# Autodesk Inventor assembly: Stadio6
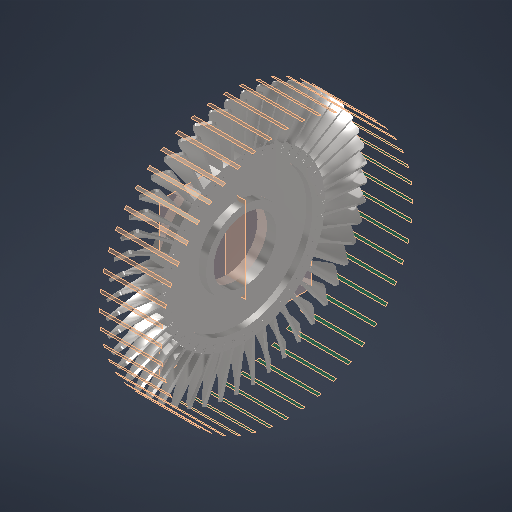
[picture p0: Inventor's stored thumbnail of the model, 512x512]
Saved by Autodesk Inventor 2026.2 (Build 302298010, 298A)
## iProperties
Created: 2026-04-24
Part Number: Stadio6
Document SubType Name: Assembly
Designer: Yan
Author: Yan
## Documents named in this file (3)
- C:\Users\Yan\Desktop\Turbina\Stadio6.iam
- C:\Users\Yan\Desktop\Turbina\DiscoPaleStadio6-DimensioniAprossimate.ipt
- C:\Users\Yan\Desktop\Turbina\PalaStadio6.ipt
## Components (49 placed, 2 different names)
1. DiscoPaleStadio6-DimensioniAprossimate:1 — Mate:1, Mate:2, Mate:3, Mate:4, Mate:5, Mate:6, Mate:7, Mate:8, Mate:9, Mate:10, Mate:11, Mate:12, Mate:13, Mate:14, Mate:15, Mate:16, Mate:17, Mate:18, Mate:19, Mate:20, Mate:21, Mate:22, Mate:24, Mate:25, Mate:26, Mate:27, Mate:28, Mate:29, Mate:30, Mate:31, Mate:32, Mate:33, Mate:34, Mate:35, Mate:36, Mate:37, Mate:38, Mate:39, Mate:40, Mate:41, Mate:42, Mate:43, Mate:44, Mate:45, Mate:46, Mate:47, Mate:48, Mate:49, Mate:50, Mate:51, Mate:52, Mate:53, Mate:56, Mate:57, Mate:58, Mate:59, Mate:60, Mate:61, Mate:62, Mate:63, Mate:64, Mate:65, Mate:66, Mate:67, Mate:68, Mate:69, Mate:70, Mate:71, Mate:72, Mate:73, Mate:74, Mate:75, Mate:76, Mate:77, Mate:78, Mate:79, Mate:80, Mate:81, Mate:82, Mate:83, Mate:84, Mate:85, Mate:86, Mate:87, Mate:88, Mate:89, Mate:90, Mate:91, Mate:92, Mate:93, Mate:94, Mate:95, Mate:96, Mate:97, Mate:98, Flush:1, Flush:2, Flush:3, Flush:4, Flush:5, Flush:6, Flush:7, Flush:8, Flush:9, Flush:10, Flush:11, Flush:12, Flush:13, Flush:14, Flush:15, Flush:16, Flush:17, Flush:18, Flush:19, Flush:20, Flush:21, Flush:22, Flush:23, Flush:24, Flush:25, Flush:26, Flush:27, Flush:28, Flush:29, Flush:30, Flush:31, Flush:32, Flush:33, Flush:34, Flush:35, Flush:36, Flush:37, Flush:38, Flush:39, Flush:40, Flush:41, Flush:42, Flush:43, Flush:44, Flush:45, Flush:46, Flush:47, Flush:48, Mate:99, Mate:100
2. PalaStadio6:1 — Mate:1, Mate:28, Flush:30
3. PalaStadio6:2 — Mate:2, Mate:27, Flush:29
4. PalaStadio6:3 — Mate:3, Mate:76, Mate:77, Flush:28
5. PalaStadio6:4 — Mate:4, Mate:29, Flush:27
6. PalaStadio6:5 — Mate:5, Mate:30, Flush:26
7. PalaStadio6:6 — Mate:7, Mate:32, Flush:24
8. PalaStadio6:7 — Mate:8, Mate:33, Flush:23
9. PalaStadio6:8 — Mate:9, Mate:34, Flush:22
10. PalaStadio6:9 — Mate:10, Mate:35, Flush:21
11. PalaStadio6:10 — Mate:11, Mate:36, Flush:20
12. PalaStadio6:11 — Mate:12, Mate:37, Flush:19
13. PalaStadio6:12 — Mate:13, Mate:38, Flush:18
14. PalaStadio6:13 — Mate:68, Mate:81, Flush:36
15. PalaStadio6:14 — Mate:6, Mate:31, Flush:25
16. PalaStadio6:15 — Mate:48, Mate:49, Flush:8
17. PalaStadio6:16 — Mate:22, Mate:47, Flush:9
18. PalaStadio6:17 — Mate:21, Mate:46, Flush:10
19. PalaStadio6:18 — Mate:20, Mate:45, Flush:11
20. PalaStadio6:19 — Mate:19, Mate:44, Flush:12
21. PalaStadio6:20 — Mate:18, Mate:43, Flush:13
22. PalaStadio6:21 — Mate:17, Mate:42, Flush:14
23. PalaStadio6:22 — Mate:16, Mate:41, Flush:15
24. PalaStadio6:23 — Mate:15, Mate:40, Flush:16
25. PalaStadio6:24 — Mate:14, Mate:39, Flush:17
26. PalaStadio6:25 — Mate:60, Mate:91, Flush:45
27. PalaStadio6:26 — Mate:59, Mate:92, Flush:46
28. PalaStadio6:27 — Mate:87, Flush:42
29. PalaStadio6:28 — Mate:58, Mate:93, Flush:47
30. PalaStadio6:29 — Mate:57, Mate:94, Flush:48
31. PalaStadio6:30 — Mate:56, Mate:95, Flush:2
32. PalaStadio6:31 — Mate:97, Flush:1, Mate:100
33. PalaStadio6:32 — Mate:98, Flush:3, Mate:99
34. PalaStadio6:33 — Mate:53, Mate:96, Flush:4
35. PalaStadio6:34 — Mate:26, Mate:52, Flush:5
36. PalaStadio6:35 — Mate:25, Mate:51, Flush:6
37. PalaStadio6:36 — Mate:24, Mate:50, Flush:7
38. PalaStadio6:37 — Mate:72, Mate:75, Flush:32
39. PalaStadio6:38 — Mate:73, Mate:74, Flush:31
40. PalaStadio6:39 — Mate:70, Mate:79, Flush:34
41. PalaStadio6:40 — Mate:71, Mate:78, Flush:33
42. PalaStadio6:41 — Mate:69, Mate:80, Flush:35
43. PalaStadio6:42 — Mate:67, Mate:82, Flush:37
44. PalaStadio6:43 — Mate:66, Mate:83, Flush:38
45. PalaStadio6:44 — Mate:65, Mate:84, Flush:39
46. PalaStadio6:45 — Mate:64, Mate:85, Mate:88, Flush:40
47. PalaStadio6:46 — Mate:63, Mate:86, Flush:41
48. PalaStadio6:47 — Mate:62, Mate:89, Flush:43
49. PalaStadio6:48 — Mate:61, Mate:90, Flush:44
## Relationships (145: Mate 97, Flush 48)
- Mate:1: DiscoPaleStadio6-DimensioniAprossimate:1 ↔ PalaStadio6:1
- Mate:2: DiscoPaleStadio6-DimensioniAprossimate:1 ↔ PalaStadio6:2
- Mate:3: DiscoPaleStadio6-DimensioniAprossimate:1 ↔ PalaStadio6:3
- Mate:4: DiscoPaleStadio6-DimensioniAprossimate:1 ↔ PalaStadio6:4
- Mate:5: DiscoPaleStadio6-DimensioniAprossimate:1 ↔ PalaStadio6:5
- Mate:6: DiscoPaleStadio6-DimensioniAprossimate:1 ↔ PalaStadio6:14
- Mate:7: DiscoPaleStadio6-DimensioniAprossimate:1 ↔ PalaStadio6:6
- Mate:8: DiscoPaleStadio6-DimensioniAprossimate:1 ↔ PalaStadio6:7
- Mate:9: DiscoPaleStadio6-DimensioniAprossimate:1 ↔ PalaStadio6:8
- Mate:10: DiscoPaleStadio6-DimensioniAprossimate:1 ↔ PalaStadio6:9
- Mate:11: DiscoPaleStadio6-DimensioniAprossimate:1 ↔ PalaStadio6:10
- Mate:12: DiscoPaleStadio6-DimensioniAprossimate:1 ↔ PalaStadio6:11
- Mate:13: DiscoPaleStadio6-DimensioniAprossimate:1 ↔ PalaStadio6:12
- Mate:14: DiscoPaleStadio6-DimensioniAprossimate:1 ↔ PalaStadio6:24
- Mate:15: DiscoPaleStadio6-DimensioniAprossimate:1 ↔ PalaStadio6:23
- Mate:16: DiscoPaleStadio6-DimensioniAprossimate:1 ↔ PalaStadio6:22
- Mate:17: DiscoPaleStadio6-DimensioniAprossimate:1 ↔ PalaStadio6:21
- Mate:18: DiscoPaleStadio6-DimensioniAprossimate:1 ↔ PalaStadio6:20
- Mate:19: DiscoPaleStadio6-DimensioniAprossimate:1 ↔ PalaStadio6:19
- Mate:20: DiscoPaleStadio6-DimensioniAprossimate:1 ↔ PalaStadio6:18
- Mate:21: DiscoPaleStadio6-DimensioniAprossimate:1 ↔ PalaStadio6:17
- Mate:22: DiscoPaleStadio6-DimensioniAprossimate:1 ↔ PalaStadio6:16
- Mate:24: DiscoPaleStadio6-DimensioniAprossimate:1 ↔ PalaStadio6:36
- Mate:25: DiscoPaleStadio6-DimensioniAprossimate:1 ↔ PalaStadio6:35
- Mate:26: DiscoPaleStadio6-DimensioniAprossimate:1 ↔ PalaStadio6:34
- Mate:27: DiscoPaleStadio6-DimensioniAprossimate:1 ↔ PalaStadio6:2
- Mate:28: DiscoPaleStadio6-DimensioniAprossimate:1 ↔ PalaStadio6:1
- Mate:29: DiscoPaleStadio6-DimensioniAprossimate:1 ↔ PalaStadio6:4
- Mate:30: DiscoPaleStadio6-DimensioniAprossimate:1 ↔ PalaStadio6:5
- Mate:31: DiscoPaleStadio6-DimensioniAprossimate:1 ↔ PalaStadio6:14
- Mate:32: DiscoPaleStadio6-DimensioniAprossimate:1 ↔ PalaStadio6:6
- Mate:33: DiscoPaleStadio6-DimensioniAprossimate:1 ↔ PalaStadio6:7
- Mate:34: DiscoPaleStadio6-DimensioniAprossimate:1 ↔ PalaStadio6:8
- Mate:35: DiscoPaleStadio6-DimensioniAprossimate:1 ↔ PalaStadio6:9
- Mate:36: DiscoPaleStadio6-DimensioniAprossimate:1 ↔ PalaStadio6:10
- Mate:37: DiscoPaleStadio6-DimensioniAprossimate:1 ↔ PalaStadio6:11
- Mate:38: DiscoPaleStadio6-DimensioniAprossimate:1 ↔ PalaStadio6:12
- Mate:39: DiscoPaleStadio6-DimensioniAprossimate:1 ↔ PalaStadio6:24
- Mate:40: DiscoPaleStadio6-DimensioniAprossimate:1 ↔ PalaStadio6:23
- Mate:41: DiscoPaleStadio6-DimensioniAprossimate:1 ↔ PalaStadio6:22
- Mate:42: DiscoPaleStadio6-DimensioniAprossimate:1 ↔ PalaStadio6:21
- Mate:43: DiscoPaleStadio6-DimensioniAprossimate:1 ↔ PalaStadio6:20
- Mate:44: DiscoPaleStadio6-DimensioniAprossimate:1 ↔ PalaStadio6:19
- Mate:45: DiscoPaleStadio6-DimensioniAprossimate:1 ↔ PalaStadio6:18
- Mate:46: DiscoPaleStadio6-DimensioniAprossimate:1 ↔ PalaStadio6:17
- Mate:47: DiscoPaleStadio6-DimensioniAprossimate:1 ↔ PalaStadio6:16
- Mate:48: DiscoPaleStadio6-DimensioniAprossimate:1 ↔ PalaStadio6:15
- Mate:49: DiscoPaleStadio6-DimensioniAprossimate:1 ↔ PalaStadio6:15
- Mate:50: DiscoPaleStadio6-DimensioniAprossimate:1 ↔ PalaStadio6:36
- Mate:51: DiscoPaleStadio6-DimensioniAprossimate:1 ↔ PalaStadio6:35
- Mate:52: DiscoPaleStadio6-DimensioniAprossimate:1 ↔ PalaStadio6:34
- Mate:53: DiscoPaleStadio6-DimensioniAprossimate:1 ↔ PalaStadio6:33
- Mate:56: DiscoPaleStadio6-DimensioniAprossimate:1 ↔ PalaStadio6:30
- Mate:57: DiscoPaleStadio6-DimensioniAprossimate:1 ↔ PalaStadio6:29
- Mate:58: DiscoPaleStadio6-DimensioniAprossimate:1 ↔ PalaStadio6:28
- Mate:59: DiscoPaleStadio6-DimensioniAprossimate:1 ↔ PalaStadio6:26
- Mate:60: DiscoPaleStadio6-DimensioniAprossimate:1 ↔ PalaStadio6:25
- Mate:61: DiscoPaleStadio6-DimensioniAprossimate:1 ↔ PalaStadio6:48
- Mate:62: DiscoPaleStadio6-DimensioniAprossimate:1 ↔ PalaStadio6:47
- Mate:63: DiscoPaleStadio6-DimensioniAprossimate:1 ↔ PalaStadio6:46
- Mate:64: DiscoPaleStadio6-DimensioniAprossimate:1 ↔ PalaStadio6:45
- Mate:65: DiscoPaleStadio6-DimensioniAprossimate:1 ↔ PalaStadio6:44
- Mate:66: DiscoPaleStadio6-DimensioniAprossimate:1 ↔ PalaStadio6:43
- Mate:67: DiscoPaleStadio6-DimensioniAprossimate:1 ↔ PalaStadio6:42
- Mate:68: DiscoPaleStadio6-DimensioniAprossimate:1 ↔ PalaStadio6:13
- Mate:69: DiscoPaleStadio6-DimensioniAprossimate:1 ↔ PalaStadio6:41
- Mate:70: DiscoPaleStadio6-DimensioniAprossimate:1 ↔ PalaStadio6:39
- Mate:71: DiscoPaleStadio6-DimensioniAprossimate:1 ↔ PalaStadio6:40
- Mate:72: DiscoPaleStadio6-DimensioniAprossimate:1 ↔ PalaStadio6:37
- Mate:73: DiscoPaleStadio6-DimensioniAprossimate:1 ↔ PalaStadio6:38
- Mate:74: DiscoPaleStadio6-DimensioniAprossimate:1 ↔ PalaStadio6:38
- Mate:75: DiscoPaleStadio6-DimensioniAprossimate:1 ↔ PalaStadio6:37
- Mate:76: DiscoPaleStadio6-DimensioniAprossimate:1 ↔ PalaStadio6:3
- Mate:77: DiscoPaleStadio6-DimensioniAprossimate:1 ↔ PalaStadio6:3
- Mate:78: DiscoPaleStadio6-DimensioniAprossimate:1 ↔ PalaStadio6:40
- Mate:79: DiscoPaleStadio6-DimensioniAprossimate:1 ↔ PalaStadio6:39
- Mate:80: DiscoPaleStadio6-DimensioniAprossimate:1 ↔ PalaStadio6:41
- Mate:81: DiscoPaleStadio6-DimensioniAprossimate:1 ↔ PalaStadio6:13
- Mate:82: DiscoPaleStadio6-DimensioniAprossimate:1 ↔ PalaStadio6:42
- Mate:83: DiscoPaleStadio6-DimensioniAprossimate:1 ↔ PalaStadio6:43
- Mate:84: DiscoPaleStadio6-DimensioniAprossimate:1 ↔ PalaStadio6:44
- Mate:85: DiscoPaleStadio6-DimensioniAprossimate:1 ↔ PalaStadio6:45
- Mate:86: DiscoPaleStadio6-DimensioniAprossimate:1 ↔ PalaStadio6:46
- Mate:87: DiscoPaleStadio6-DimensioniAprossimate:1 ↔ PalaStadio6:27
- Mate:88: DiscoPaleStadio6-DimensioniAprossimate:1 ↔ PalaStadio6:45
- Mate:89: DiscoPaleStadio6-DimensioniAprossimate:1 ↔ PalaStadio6:47
- Mate:90: DiscoPaleStadio6-DimensioniAprossimate:1 ↔ PalaStadio6:48
- Mate:91: DiscoPaleStadio6-DimensioniAprossimate:1 ↔ PalaStadio6:25
- Mate:92: DiscoPaleStadio6-DimensioniAprossimate:1 ↔ PalaStadio6:26
- Mate:93: DiscoPaleStadio6-DimensioniAprossimate:1 ↔ PalaStadio6:28
- Mate:94: DiscoPaleStadio6-DimensioniAprossimate:1 ↔ PalaStadio6:29
- Mate:95: DiscoPaleStadio6-DimensioniAprossimate:1 ↔ PalaStadio6:30
- Mate:96: DiscoPaleStadio6-DimensioniAprossimate:1 ↔ PalaStadio6:33
- Mate:97: DiscoPaleStadio6-DimensioniAprossimate:1 ↔ PalaStadio6:31
- Mate:98: DiscoPaleStadio6-DimensioniAprossimate:1 ↔ PalaStadio6:32
- Flush:1: DiscoPaleStadio6-DimensioniAprossimate:1 ↔ PalaStadio6:31
- Flush:2: DiscoPaleStadio6-DimensioniAprossimate:1 ↔ PalaStadio6:30
- Flush:3: DiscoPaleStadio6-DimensioniAprossimate:1 ↔ PalaStadio6:32
- Flush:4: DiscoPaleStadio6-DimensioniAprossimate:1 ↔ PalaStadio6:33
- Flush:5: DiscoPaleStadio6-DimensioniAprossimate:1 ↔ PalaStadio6:34
- Flush:6: DiscoPaleStadio6-DimensioniAprossimate:1 ↔ PalaStadio6:35
- Flush:7: DiscoPaleStadio6-DimensioniAprossimate:1 ↔ PalaStadio6:36
- Flush:8: DiscoPaleStadio6-DimensioniAprossimate:1 ↔ PalaStadio6:15
- Flush:9: DiscoPaleStadio6-DimensioniAprossimate:1 ↔ PalaStadio6:16
- Flush:10: DiscoPaleStadio6-DimensioniAprossimate:1 ↔ PalaStadio6:17
- Flush:11: DiscoPaleStadio6-DimensioniAprossimate:1 ↔ PalaStadio6:18
- Flush:12: DiscoPaleStadio6-DimensioniAprossimate:1 ↔ PalaStadio6:19
- Flush:13: DiscoPaleStadio6-DimensioniAprossimate:1 ↔ PalaStadio6:20
- Flush:14: DiscoPaleStadio6-DimensioniAprossimate:1 ↔ PalaStadio6:21
- Flush:15: DiscoPaleStadio6-DimensioniAprossimate:1 ↔ PalaStadio6:22
- Flush:16: DiscoPaleStadio6-DimensioniAprossimate:1 ↔ PalaStadio6:23
- Flush:17: DiscoPaleStadio6-DimensioniAprossimate:1 ↔ PalaStadio6:24
- Flush:18: DiscoPaleStadio6-DimensioniAprossimate:1 ↔ PalaStadio6:12
- Flush:19: DiscoPaleStadio6-DimensioniAprossimate:1 ↔ PalaStadio6:11
- Flush:20: DiscoPaleStadio6-DimensioniAprossimate:1 ↔ PalaStadio6:10
- Flush:21: DiscoPaleStadio6-DimensioniAprossimate:1 ↔ PalaStadio6:9
- Flush:22: DiscoPaleStadio6-DimensioniAprossimate:1 ↔ PalaStadio6:8
- Flush:23: DiscoPaleStadio6-DimensioniAprossimate:1 ↔ PalaStadio6:7
- Flush:24: DiscoPaleStadio6-DimensioniAprossimate:1 ↔ PalaStadio6:6
- Flush:25: DiscoPaleStadio6-DimensioniAprossimate:1 ↔ PalaStadio6:14
- Flush:26: DiscoPaleStadio6-DimensioniAprossimate:1 ↔ PalaStadio6:5
- Flush:27: DiscoPaleStadio6-DimensioniAprossimate:1 ↔ PalaStadio6:4
- Flush:28: DiscoPaleStadio6-DimensioniAprossimate:1 ↔ PalaStadio6:3
- Flush:29: DiscoPaleStadio6-DimensioniAprossimate:1 ↔ PalaStadio6:2
- Flush:30: DiscoPaleStadio6-DimensioniAprossimate:1 ↔ PalaStadio6:1
- Flush:31: DiscoPaleStadio6-DimensioniAprossimate:1 ↔ PalaStadio6:38
- Flush:32: DiscoPaleStadio6-DimensioniAprossimate:1 ↔ PalaStadio6:37
- Flush:33: DiscoPaleStadio6-DimensioniAprossimate:1 ↔ PalaStadio6:40
- Flush:34: DiscoPaleStadio6-DimensioniAprossimate:1 ↔ PalaStadio6:39
- Flush:35: DiscoPaleStadio6-DimensioniAprossimate:1 ↔ PalaStadio6:41
- Flush:36: DiscoPaleStadio6-DimensioniAprossimate:1 ↔ PalaStadio6:13
- Flush:37: DiscoPaleStadio6-DimensioniAprossimate:1 ↔ PalaStadio6:42
- Flush:38: DiscoPaleStadio6-DimensioniAprossimate:1 ↔ PalaStadio6:43
- Flush:39: DiscoPaleStadio6-DimensioniAprossimate:1 ↔ PalaStadio6:44
- Flush:40: DiscoPaleStadio6-DimensioniAprossimate:1 ↔ PalaStadio6:45
- Flush:41: DiscoPaleStadio6-DimensioniAprossimate:1 ↔ PalaStadio6:46
- Flush:42: DiscoPaleStadio6-DimensioniAprossimate:1 ↔ PalaStadio6:27
- Flush:43: DiscoPaleStadio6-DimensioniAprossimate:1 ↔ PalaStadio6:47
- Flush:44: DiscoPaleStadio6-DimensioniAprossimate:1 ↔ PalaStadio6:48
- Flush:45: DiscoPaleStadio6-DimensioniAprossimate:1 ↔ PalaStadio6:25
- Flush:46: DiscoPaleStadio6-DimensioniAprossimate:1 ↔ PalaStadio6:26
- Flush:47: DiscoPaleStadio6-DimensioniAprossimate:1 ↔ PalaStadio6:28
- Flush:48: DiscoPaleStadio6-DimensioniAprossimate:1 ↔ PalaStadio6:29
- Mate:99: DiscoPaleStadio6-DimensioniAprossimate:1 ↔ PalaStadio6:32
- Mate:100: DiscoPaleStadio6-DimensioniAprossimate:1 ↔ PalaStadio6:31
